# Autodesk Inventor assembly: hubRings
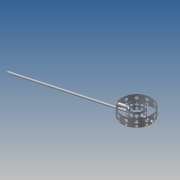
[picture p0: Inventor's stored thumbnail of the model, 180x180]
Saved by Autodesk Inventor 2014 SP1 (Build 180222100, 222)
## iProperties
Created: 2014-12-05
Part Number: hubRings
Document SubType Name: Assembly
Designer: Dave
Author: Dave
## Documents named in this file (9)
- C:\Users\Dave\Desktop\hera-cad\hub\hubRings.iam
- C:\Users\Dave\Desktop\hera-cad\hub\ringOuter_Split.ipt
- C:\Users\Dave\Desktop\hera-cad\hub\ringOuter_Split_MIR.ipt
- C:\Users\Dave\Desktop\hera-cad\hub\hubGuideRingOuter.ipt
- C:\Users\Dave\Desktop\hera-cad\hub\ringInner.ipt
- C:\Users\Dave\Desktop\hera-cad\hub\hubGuideRingInner.ipt
- C:\Users\Dave\Desktop\hera-cad\hub\sleeve_spar.ipt
- C:\Users\Dave\Desktop\hera-cad\hub\conduit.ipt
- C:\Users\Dave\Desktop\hera-cad\support\sparHoriz.ipt
## Components (8 placed, 8 different names)
1. ringOuter_Split:1 — Flush:1, Insert:2
2. ringOuter_Split_MIR:1 — Flush:1, Flush:2
3. hubGuideRingOuter:1 — Insert:1, Insert:2, Insert:3, Insert:4
4. ringInner:1 — Flush:2
5. hubGuideRingInner:1 — Insert:1
6. sleeve_spar:1 — Insert:3
7. conduit:1
8. sparHoriz:1 — Insert:4
## Relationships (6: Insert 4, Flush 2)
- Flush:1: ringOuter_Split:1 ↔ ringOuter_Split_MIR:1
- Insert:1: hubGuideRingOuter:1 ↔ hubGuideRingInner:1
- Flush:2: ringOuter_Split_MIR:1 ↔ ringInner:1
- Insert:2: ringOuter_Split:1 ↔ hubGuideRingOuter:1
- Insert:3 (-260.35 mm): hubGuideRingOuter:1 ↔ sleeve_spar:1
- Insert:4 (-260.35 mm): hubGuideRingOuter:1 ↔ sparHoriz:1
